# Autodesk Inventor assembly: Arm 2.0 Assembly
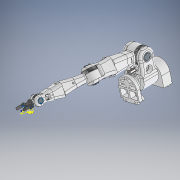
[picture p0: Inventor's stored thumbnail of the model, 180x180]
Saved by Autodesk Inventor 2017 SP1 (Build 210196100, 196)
## iProperties
Created: 2017-09-28
Part Number: Arm 2.0 Assembly
Document SubType Name: Assembly
Designer: Zach
Author: Zach
## Documents named in this file (43)
- C:\Users\Zach\Documents\GitHub\tr1\src\Body\Arm 2.0 Assembly\Arm 2.0 Assembly.iam
- C:\Users\Zach\Documents\GitHub\tr1\src\Body\Arm 2.0 Assembly\Steel Rod 8mm x 135mm.ipt
- C:\Users\Zach\Documents\GitHub\tr1\lib\22x8x8mm Bearing.ipt
- C:\Users\Zach\Documents\GitHub\tr1\src\Body\Arm 2.0 Assembly\AA004.ipt
- C:\Users\Zach\Documents\GitHub\tr1\lib\QS12MM250\QS12MM250.ipt
- C:\Users\Zach\Documents\GitHub\tr1\src\Body\Arm 2.0 Assembly\AA010.ipt
- C:\Users\Zach\Documents\GitHub\tr1\src\Body\Arm 2.0 Assembly\Steel Rod 8mm x 100mm.ipt
- C:\Users\Zach\Documents\GitHub\tr1\src\Body\Arm 2.0 Assembly\AA013.ipt
- C:\Users\Zach\Documents\GitHub\tr1\src\Body\Arm 2.0 Assembly\AA014.ipt
- C:\Users\Zach\Documents\GitHub\tr1\lib\12V DC Motor 378-1.ipt
- C:\Users\Zach\Documents\Inventor\Content Center Files\R2017\en-US\ISO 4016\ISO 4016 - M5 x 25.ipt
- C:\Users\Zach\Documents\Inventor\Content Center Files\R2017\en-US\ISO 4017(1)\ISO 4017 - M5 x 12 - ISO.ipt
- C:\Users\Zach\Documents\Inventor\Content Center Files\R2017\en-US\ISO 4017(1)\ISO 4017 - M5 x 20 - ISO.ipt
- C:\Users\Zach\Documents\GitHub\tr1\src\Body\Arm 2.0 Assembly\AA019.ipt
- C:\Users\Zach\Documents\GitHub\tr1\src\Body\Arm 2.0 Assembly\AA020.ipt
- C:\Users\Zach\Documents\GitHub\tr1\src\Body\Arm 2.0 Assembly\AA021.ipt
- C:\Users\Zach\Documents\GitHub\tr1\src\Body\Arm 2.0 Assembly\Steel Rod 8mm x 80mm.ipt
- C:\Users\Zach\Documents\GitHub\tr1\src\Body\Arm 2.0 Assembly\AA023.ipt
- C:\Users\Zach\Documents\GitHub\BCN3D-Moveo\Autodesk Inventor files\Gripper B Assembly.iam
- C:\Users\Zach\Documents\Inventor\Content Center Files\R2017\en-US\CNS 4320\CNS 4320 - M8 x 1 x 100.ipt
- C:\Users\Zach\Documents\GitHub\tr1\lib\AS 1110 - M8 x 150.ipt
- C:\Users\Zach\Documents\GitHub\tr1\lib\8mm Hub.ipt
- C:\Users\Zach\Documents\GitHub\tr1\src\Body\Arm 2.0 Assembly\Arm 2.0 Assembly\Design Accelerator\Spur Gears5.iam
- C:\Users\Zach\Documents\GitHub\tr1\lib\4mm mounting hub.ipt
- C:\Users\Zach\Documents\GitHub\tr1\lib\6201RS\6201RS.ipt
- C:\Users\Zach\Documents\GitHub\tr1\lib\U51105\U51105.ipt
- C:\Users\Zach\Documents\GitHub\tr1\src\Body\Arm 2.0 Assembly\AA033.ipt
- C:\Users\Zach\Documents\GitHub\tr1\src\Body\Arm 2.0 Assembly\AA032.ipt
- C:\Users\Zach\Documents\GitHub\tr1\src\Body\Arm 2.0 Assembly\AA031.ipt
- C:\Users\Zach\Documents\GitHub\tr1\lib\Timing Pulley - T5 4mm Bore 15mm Width.ipt
- C:\Users\Zach\Documents\GitHub\tr1\src\Body\Arm 2.0 Assembly\AA034.ipt
- C:\Users\Zach\Documents\GitHub\tr1\src\Body\Arm 2.0 Assembly\Arm 2.0 Assembly\Design Accelerator\Spur Gears6.iam
- C:\Users\Zach\Documents\GitHub\tr1\src\Body\Arm 2.0 Assembly\AA008c.ipt
- C:\Users\Zach\Documents\GitHub\tr1\src\Body\Arm 2.0 Assembly\AA008d.ipt
- C:\Users\Zach\Documents\GitHub\tr1\src\Body\Arm 2.0 Assembly\AA035.ipt
- C:\Users\Zach\Documents\GitHub\tr1\src\Body\Arm 2.0 Assembly\Arm 2.0 Assembly\Design Accelerator\Spur Gears7.iam
- C:\Users\Zach\Documents\GitHub\tr1\src\Body\Arm 2.0 Assembly\AA036.ipt
- C:\Users\Zach\Documents\GitHub\tr1\src\Body\Arm 2.0 Assembly\AA037.ipt
- C:\Users\Zach\Documents\GitHub\tr1\src\Body\Arm 2.0 Assembly\AA016b.ipt
- C:\Users\Zach\Documents\GitHub\tr1\src\Body\Arm 2.0 Assembly\AA005b.ipt
- C:\Users\Zach\Documents\GitHub\tr1\src\Body\Arm 2.0 Assembly\AA006b.ipt
- C:\Users\Zach\Documents\GitHub\tr1\src\Body\Arm 2.0 Assembly\AA001c.ipt
- C:\Users\Zach\Documents\GitHub\tr1\lib\uxcell 12V 5RPM 8mm Worm Gear Motor\uxcell 12V 5RPM 8mm Worm Gear Motor.ipt
## Components (76 placed, 40 different names)
1. AA001c:1 — Mate:554, Mate:555, Mate:556, Mate:557, Mate:558, Mate:559, Mate:560, Flush:18, Mate:561, Mate:562, Mate:563, Mate:564, Mate:565, Mate:566, Mate:567, Mate:568, Mate:569, Mate:570, Mate:571, Mate:572
2. AA004:1 — Mate:23, Mate:345, Mate:347, Mate:350, Mate:352, Mate:353, Mate:357, Mate:554, Mate:555, Mate:556
3. AA005b:1 — Mate:537, Mate:538, Mate:539, Mate:541, Mate:542, Mate:543, Mate:546
4. AA006b:1 — Mate:544, Mate:545, Mate:546
5. AA008c:1 — Mate:449, Mate:450, Mate:451, Mate:452, Mate:453, Mate:454, Mate:463, Mate:464, Mate:466, Mate:467, Mate:481, Mate:497
6. AA008d:1 — Mate:455, Mate:456, Mate:457, Mate:461, Mate:463, Mate:464, Mate:466, Mate:467, Mate:480, Mate:482
7. AA010:1 — Mate:55, Flush:6, Mate:56, Flush:7, Flush:8, Mate:64, Mate:65, Mate:66, Mate:67, Mate:68, Mate:69, Mate:486, Mate:487, Mate:488, Mate:490, Mate:492, Mate:493, Mate:494, Mate:495, Mate:496, Mate:497
8. AA013:1 — Mate:148, Mate:149, Mate:150, Mate:151, Mate:152, Mate:153, Mate:436, Mate:558, Mate:559
9. AA013:2 — Mate:142, Mate:143, Mate:144, Mate:145, Mate:146, Mate:147, Mate:563, Mate:564, Mate:565
10. AA014:1 — Mate:64, Mate:65, Mate:66, Mate:160, Mate:161, Mate:162, Mate:163, Mate:164, Mate:165
11. AA014:2 — Mate:67, Mate:68, Mate:69, Mate:154, Mate:155, Mate:156, Mate:157, Mate:158, Mate:159
12. AA016b:1 — Mate:518, Mate:519, Mate:520, Mate:521, Mate:525, Mate:526, Mate:527, Mate:529, Mate:530
13. AA019:1 — Mate:174, Mate:175, Mate:182, Mate:183, Mate:185, Flush:15, Flush:16, Flush:17, Mate:188, Mate:189, Mate:190, Mate:191, Mate:192, Mate:193, Mate:388, Mate:400, Mate:401, Mate:533, Mate:536
14. AA020:1 — Mate:171, Mate:172, Mate:173, Mate:175, Mate:194, Mate:196
15. AA021:1 — Mate:171, Mate:172, Mate:173, Mate:174, Mate:195
16. AA023:1 — Mate:188, Mate:189, Mate:193
17. AA023:2 — Mate:190, Mate:191, Mate:192
18. AA031:1 — Mate:366, Mate:367, Mate:523, Mate:524
19. AA032:2 — Mate:465
20. AA033:1 — Mate:351, Mate:352, Mate:353, Mate:355, Mate:356
21. AA034:1 — Mate:388, Mate:529, Mate:533, Mate:534, Mate:535, Mate:536
22. AA036:1 — Mate:498, Mate:500, Mate:501, Mate:502, Mate:503, Mate:511
23. AA037:1 — Mate:501, Mate:502, Mate:503, Mate:514, Mate:515, Mate:516, Mate:517, Mate:518, Mate:519, Mate:520, Mate:530
24. Gripper B Assembly:1 [sub-assembly] — Mate:194, Mate:195, Mate:196
25. 22x8x8mm Bearing:1 — Mate:433, Mate:560
26. 22x8x8mm Bearing:2 — Mate:437, Mate:562
27. 22x8x8mm Bearing:3 — Mate:55, Flush:6, Mate:57
28. 22x8x8mm Bearing:4 — Mate:56, Flush:7
29. 22x8x8mm Bearing:5 — Mate:186, Flush:16
30. 22x8x8mm Bearing:6 — Mate:187, Flush:17
31. 22x8x8mm Bearing:7 — Mate:264, Mate:526
32. 22x8x8mm Bearing:8 — Mate:527, Mate:528
33. 22x8x8mm Bearing:13 — Mate:451, Mate:452
34. 22x8x8mm Bearing:14 — Mate:449, Mate:450
35. QS12MM250:1 — Mate:23, Mate:344, Mate:346, Mate:348, Mate:351, Mate:354, Mate:484, Mate:537, Mate:544
36. Steel Rod 8mm x 135mm:1 — Mate:433, Mate:436, Mate:437, Mate:476, Mate:477, Flush:18
37. Steel Rod 8mm x 100mm:1 — Mate:57, Flush:8, Mate:491, Mate:498
38. Steel Rod 8mm x 80mm:1 — Mate:185, Flush:15, Mate:186, Mate:187
39. 12V DC Motor 378-1:2 — Mate:376, Mate:486, Mate:487, Mate:488, Mate:489
40. 12V DC Motor 378-1:3 — Mate:182, Mate:183, Mate:392, Mate:394, Mate:400
41. 12V DC Motor 378-1:4 — Mate:514, Mate:515, Mate:516, Mate:522
42. 12V DC Motor 378-1:6 — Mate:340, Mate:342, Mate:538, Mate:539, Mate:540, Mate:543
43. 12V DC Motor 378-1:7 — Mate:455, Mate:456, Mate:457, Mate:460, Mate:465
44. 6201RS:1 — Mate:346, Mate:347
45. 6201RS:2 — Mate:356, Mate:357
46. U51105:1 — Mate:348, Mate:349, Mate:542
47. U51105:2 — Mate:354, Mate:355, Mate:545
48. 8mm Hub:2 — Mate:368, Mate:531, Mate:534, Mate:535
49. 8mm Hub:3 — Mate:493, Mate:494, Mate:495
50. 4mm mounting hub:1 — Mate:340, Mate:343, Mate:540, Mate:541
51. 4mm mounting hub:3 — Mate:366, Mate:367, Mate:517, Mate:522, Mate:523, Mate:524
52. 4mm mounting hub:5 — Mate:376, Mate:513
53. 4mm mounting hub:6 — Mate:392, Mate:395, Mate:396, Mate:401
54. 4mm mounting hub:7 — Mate:460, Mate:461
55. Timing Pulley - T5 4mm Bore 15mm Width:3 — Mate:394, Mate:395, Mate:396
56. ISO 4016 M5 x 25:9
57. ISO 4016 M5 x 25:10
58. ISO 4017 M5 x 20:1 — Mate:146, Mate:147
59. ISO 4017 M5 x 20:2 — Mate:144, Mate:145
60. ISO 4017 M5 x 20:3 — Mate:142, Mate:143
61. ISO 4017 M5 x 20:4 — Mate:148, Mate:149
62. ISO 4017 M5 x 20:5 — Mate:152, Mate:153
63. ISO 4017 M5 x 20:6 — Mate:150, Mate:151
64. ISO 4017 M5 x 12:1 — Mate:154, Mate:155
65. ISO 4017 M5 x 12:2 — Mate:156, Mate:158
66. ISO 4017 M5 x 12:3 — Mate:157, Mate:159
67. ISO 4017 M5 x 12:4 — Mate:160, Mate:161
68. ISO 4017 M5 x 12:5 — Mate:162, Mate:163
69. ISO 4017 M5 x 12:6 — Mate:164, Mate:165
70. CNS 4320 M8 x 100:1 — Mate:264, Mate:368, Mate:521, Mate:525, Mate:528, Mate:531
71. AS 1110 - Metric M8 x 80:2 — Mate:453, Mate:454, Mate:496
72. Spur Gears:5 [sub-assembly] — Mate:342, Mate:343, Mate:344, Mate:345, Mate:349, Mate:350
73. Spur Gears:6 [sub-assembly] — Mate:476, Mate:478, Mate:479, Mate:566, Mate:567
74. Spur Gear2:1 — Mate:477, Mate:478, Mate:479, Mate:480, Mate:481, Mate:482, Mate:557, Mate:561
75. Spur Gears:7 [sub-assembly] — Mate:489, Mate:490, Mate:491, Mate:492, Mate:500, Mate:511, Mate:513
76. uxcell 12V 5RPM 8mm Worm Gear Motor:1 — Mate:568, Mate:569, Mate:570, Mate:571, Mate:572
## Relationships (188: Mate 181, Flush 7)
- Mate:23: AA004:1 ↔ QS12MM250:1
- Mate:55: AA010:1 ↔ 22x8x8mm Bearing:3
- Flush:6: AA010:1 ↔ 22x8x8mm Bearing:3
- Mate:56: AA010:1 ↔ 22x8x8mm Bearing:4
- Flush:7: AA010:1 ↔ 22x8x8mm Bearing:4
- Mate:57: 22x8x8mm Bearing:3 ↔ Steel Rod 8mm x 100mm:1
- Flush:8 (2.5 mm): AA010:1 ↔ Steel Rod 8mm x 100mm:1
- Mate:64: AA010:1 ↔ AA014:1
- Mate:65: AA010:1 ↔ AA014:1
- Mate:66: AA010:1 ↔ AA014:1
- Mate:67: AA010:1 ↔ AA014:2
- Mate:68: AA010:1 ↔ AA014:2
- Mate:69: AA010:1 ↔ AA014:2
- Mate:142: AA013:2 ↔ ISO 4017 M5 x 20:3
- Mate:143: AA013:2 ↔ ISO 4017 M5 x 20:3
- Mate:144: AA013:2 ↔ ISO 4017 M5 x 20:2
- Mate:145: AA013:2 ↔ ISO 4017 M5 x 20:2
- Mate:146: AA013:2 ↔ ISO 4017 M5 x 20:1
- Mate:147: AA013:2 ↔ ISO 4017 M5 x 20:1
- Mate:148: AA013:1 ↔ ISO 4017 M5 x 20:4
- Mate:149: AA013:1 ↔ ISO 4017 M5 x 20:4
- Mate:150: AA013:1 ↔ ISO 4017 M5 x 20:6
- Mate:151: AA013:1 ↔ ISO 4017 M5 x 20:6
- Mate:152: AA013:1 ↔ ISO 4017 M5 x 20:5
- Mate:153: AA013:1 ↔ ISO 4017 M5 x 20:5
- Mate:154: AA014:2 ↔ ISO 4017 M5 x 12:1
- Mate:155: AA014:2 ↔ ISO 4017 M5 x 12:1
- Mate:156: AA014:2 ↔ ISO 4017 M5 x 12:2
- Mate:157: AA014:2 ↔ ISO 4017 M5 x 12:3
- Mate:158: AA014:2 ↔ ISO 4017 M5 x 12:2
- Mate:159: AA014:2 ↔ ISO 4017 M5 x 12:3
- Mate:160: AA014:1 ↔ ISO 4017 M5 x 12:4
- Mate:161: AA014:1 ↔ ISO 4017 M5 x 12:4
- Mate:162: AA014:1 ↔ ISO 4017 M5 x 12:5
- Mate:163: AA014:1 ↔ ISO 4017 M5 x 12:5
- Mate:164: AA014:1 ↔ ISO 4017 M5 x 12:6
- Mate:165: AA014:1 ↔ ISO 4017 M5 x 12:6
- Mate:171: AA020:1 ↔ AA021:1
- Mate:172: AA020:1 ↔ AA021:1
- Mate:173: AA020:1 ↔ AA021:1
- Mate:174 (1 mm): AA019:1 ↔ AA021:1
- Mate:175: AA019:1 ↔ AA020:1
- Mate:182: AA019:1 ↔ 12V DC Motor 378-1:3
- Mate:183: AA019:1 ↔ 12V DC Motor 378-1:3
- Mate:185: AA019:1 ↔ Steel Rod 8mm x 80mm:1
- Flush:15: AA019:1 ↔ Steel Rod 8mm x 80mm:1
- Mate:186: 22x8x8mm Bearing:5 ↔ Steel Rod 8mm x 80mm:1
- Flush:16: AA019:1 ↔ 22x8x8mm Bearing:5
- Mate:187: 22x8x8mm Bearing:6 ↔ Steel Rod 8mm x 80mm:1
- Flush:17: AA019:1 ↔ 22x8x8mm Bearing:6
- Mate:188: AA019:1 ↔ AA023:1
- Mate:189: AA019:1 ↔ AA023:1
- Mate:190: AA019:1 ↔ AA023:2
- Mate:191: AA019:1 ↔ AA023:2
- Mate:192: AA019:1 ↔ AA023:2
- Mate:193: AA019:1 ↔ AA023:1
- Mate:194: AA020:1 ↔ Gripper B Assembly:1
- Mate:195: AA021:1 ↔ Gripper B Assembly:1
- Mate:196: AA020:1 ↔ Gripper B Assembly:1
- Mate:264: 22x8x8mm Bearing:7 ↔ CNS 4320 M8 x 100:1
- Mate:340: 12V DC Motor 378-1:6 ↔ 4mm mounting hub:1
- Mate:342: 12V DC Motor 378-1:6 ↔ Spur Gears:5
- Mate:343: 4mm mounting hub:1 ↔ Spur Gears:5
- Mate:344: QS12MM250:1 ↔ Spur Gears:5
- Mate:345: AA004:1 ↔ Spur Gears:5
- Mate:346: QS12MM250:1 ↔ 6201RS:1
- Mate:347: AA004:1 ↔ 6201RS:1
- Mate:348: QS12MM250:1 ↔ U51105:1
- Mate:349: U51105:1 ↔ Spur Gears:5
- Mate:350: AA004:1 ↔ Spur Gears:5
- Mate:351: AA033:1 ↔ QS12MM250:1
- Mate:352: AA004:1 ↔ AA033:1
- Mate:353: AA004:1 ↔ AA033:1
- Mate:354: QS12MM250:1 ↔ U51105:2
- Mate:355: AA033:1 ↔ U51105:2
- Mate:356: AA033:1 ↔ 6201RS:2
- Mate:357: AA004:1 ↔ 6201RS:2
- Mate:366: AA031:1 ↔ 4mm mounting hub:3
- Mate:367: AA031:1 ↔ 4mm mounting hub:3
- Mate:368: 8mm Hub:2 ↔ CNS 4320 M8 x 100:1
- Mate:376: 12V DC Motor 378-1:2 ↔ 4mm mounting hub:5
- Mate:388: AA019:1 ↔ AA034:1
- Mate:392: 12V DC Motor 378-1:3 ↔ 4mm mounting hub:6
- Mate:394: 12V DC Motor 378-1:3 ↔ Timing Pulley - T5 4mm Bore 15mm Width:3
- Mate:395: 4mm mounting hub:6 ↔ Timing Pulley - T5 4mm Bore 15mm Width:3
- Mate:396: 4mm mounting hub:6 ↔ Timing Pulley - T5 4mm Bore 15mm Width:3
- Mate:400: AA019:1 ↔ 12V DC Motor 378-1:3
- Mate:401: AA019:1 ↔ 4mm mounting hub:6
- Mate:433: 22x8x8mm Bearing:1 ↔ Steel Rod 8mm x 135mm:1
- Mate:436: AA013:1 ↔ Steel Rod 8mm x 135mm:1
- Mate:437: 22x8x8mm Bearing:2 ↔ Steel Rod 8mm x 135mm:1
- Mate:449: AA008c:1 ↔ 22x8x8mm Bearing:14
- Mate:450: AA008c:1 ↔ 22x8x8mm Bearing:14
- Mate:451: AA008c:1 ↔ 22x8x8mm Bearing:13
- Mate:452: AA008c:1 ↔ 22x8x8mm Bearing:13
- Mate:453: AA008c:1 ↔ AS 1110 - Metric M8 x 80:2
- Mate:454: AA008c:1 ↔ AS 1110 - Metric M8 x 80:2
- Mate:455: AA008d:1 ↔ 12V DC Motor 378-1:7
- Mate:456: AA008d:1 ↔ 12V DC Motor 378-1:7
- Mate:457: AA008d:1 ↔ 12V DC Motor 378-1:7
- [Mate]: AA032:2 ↔ 4mm mounting hub:7
- [Mate]: AA032:2 ↔ 4mm mounting hub:7
- Mate:460: 12V DC Motor 378-1:7 ↔ 4mm mounting hub:7
- Mate:461: AA008d:1 ↔ 4mm mounting hub:7
- Mate:463: AA008c:1 ↔ AA008d:1
- Mate:464: AA008c:1 ↔ AA008d:1
- Mate:465: AA032:2 ↔ 12V DC Motor 378-1:7
- Mate:466: AA008c:1 ↔ AA008d:1
- Mate:467: AA008c:1 ↔ AA008d:1
- Mate:476: Steel Rod 8mm x 135mm:1 ↔ Spur Gears:6
- Mate:477: Steel Rod 8mm x 135mm:1 ↔ Spur Gear2:1
- Mate:478: Spur Gears:6 ↔ Spur Gear2:1
- Mate:479: Spur Gears:6 ↔ Spur Gear2:1
- Mate:480: AA008d:1 ↔ Spur Gear2:1
- Mate:481: AA008c:1 ↔ Spur Gear2:1
- Mate:482: AA008d:1 ↔ Spur Gear2:1
- Mate:484: QS12MM250:1
- Mate:486: AA010:1 ↔ 12V DC Motor 378-1:2
- Mate:487: AA010:1 ↔ 12V DC Motor 378-1:2
- Mate:488: AA010:1 ↔ 12V DC Motor 378-1:2
- Mate:489: 12V DC Motor 378-1:2 ↔ Spur Gears:7
- Mate:490: AA010:1 ↔ Spur Gears:7
- Mate:491: Steel Rod 8mm x 100mm:1 ↔ Spur Gears:7
- Mate:492: AA010:1 ↔ Spur Gears:7
- Mate:493: AA010:1 ↔ 8mm Hub:3
- Mate:494: AA010:1 ↔ 8mm Hub:3
- Mate:495: AA010:1 ↔ 8mm Hub:3
- Mate:496: AA010:1 ↔ AS 1110 - Metric M8 x 80:2
- Mate:497: AA008c:1 ↔ AA010:1
- Mate:498: AA036:1 ↔ Steel Rod 8mm x 100mm:1
- Mate:500: AA036:1 ↔ Spur Gears:7
- Mate:501: AA036:1 ↔ AA037:1
- Mate:502: AA036:1 ↔ AA037:1
- Mate:503: AA036:1 ↔ AA037:1
- Mate:511: AA036:1 ↔ Spur Gears:7
- Mate:513: 4mm mounting hub:5 ↔ Spur Gears:7
- Mate:514: AA037:1 ↔ 12V DC Motor 378-1:4
- Mate:515: AA037:1 ↔ 12V DC Motor 378-1:4
- Mate:516: AA037:1 ↔ 12V DC Motor 378-1:4
- Mate:517: AA037:1 ↔ 4mm mounting hub:3
- Mate:518: AA016b:1 ↔ AA037:1
- Mate:519: AA016b:1 ↔ AA037:1
- Mate:520: AA016b:1 ↔ AA037:1
- Mate:521: AA016b:1 ↔ CNS 4320 M8 x 100:1
- Mate:522: 12V DC Motor 378-1:4 ↔ 4mm mounting hub:3
- Mate:523: AA031:1 ↔ 4mm mounting hub:3
- Mate:524: AA031:1 ↔ 4mm mounting hub:3
- Mate:525: AA016b:1 ↔ CNS 4320 M8 x 100:1
- Mate:526 (0.5 mm): AA016b:1 ↔ 22x8x8mm Bearing:7
- Mate:527 (0.5 mm): AA016b:1 ↔ 22x8x8mm Bearing:8
- Mate:528: 22x8x8mm Bearing:8 ↔ CNS 4320 M8 x 100:1
- Mate:529: AA016b:1 ↔ AA034:1
- Mate:530: AA016b:1 ↔ AA037:1
- Mate:531: 8mm Hub:2 ↔ CNS 4320 M8 x 100:1
- Mate:533: AA019:1 ↔ AA034:1
- Mate:534: AA034:1 ↔ 8mm Hub:2
- Mate:535: AA034:1 ↔ 8mm Hub:2
- Mate:536: AA019:1 ↔ AA034:1
- Mate:537: AA005b:1 ↔ QS12MM250:1
- Mate:538: AA005b:1 ↔ 12V DC Motor 378-1:6
- Mate:539: AA005b:1 ↔ 12V DC Motor 378-1:6
- Mate:540: 12V DC Motor 378-1:6 ↔ 4mm mounting hub:1
- Mate:541: AA005b:1 ↔ 4mm mounting hub:1
- Mate:542: AA005b:1 ↔ U51105:1
- Mate:543: AA005b:1 ↔ 12V DC Motor 378-1:6
- Mate:544: AA006b:1 ↔ QS12MM250:1
- Mate:545: AA006b:1 ↔ U51105:2
- Mate:546: AA005b:1 ↔ AA006b:1
- Mate:554: AA001c:1 ↔ AA004:1
- Mate:555: AA001c:1 ↔ AA004:1
- Mate:556: AA001c:1 ↔ AA004:1
- Mate:557: AA001c:1 ↔ Spur Gear2:1
- Mate:558: AA001c:1 ↔ AA013:1
- Mate:559: AA001c:1 ↔ AA013:1
- Mate:560: AA001c:1 ↔ 22x8x8mm Bearing:1
- Flush:18: AA001c:1 ↔ Steel Rod 8mm x 135mm:1
- Mate:561 (2.25 mm): AA001c:1 ↔ Spur Gear2:1
- Mate:562: AA001c:1 ↔ 22x8x8mm Bearing:2
- Mate:563: AA001c:1 ↔ AA013:2
- Mate:564: AA001c:1 ↔ AA013:2
- Mate:565: AA001c:1 ↔ AA013:2
- Mate:566: AA001c:1 ↔ Spur Gears:6
- Mate:567 (1 mm): AA001c:1 ↔ Spur Gears:6
- Mate:568: AA001c:1 ↔ uxcell 12V 5RPM 8mm Worm Gear Motor:1
- Mate:569: AA001c:1 ↔ uxcell 12V 5RPM 8mm Worm Gear Motor:1
- Mate:570: AA001c:1 ↔ uxcell 12V 5RPM 8mm Worm Gear Motor:1
- Mate:571: AA001c:1 ↔ uxcell 12V 5RPM 8mm Worm Gear Motor:1
- Mate:572: AA001c:1 ↔ uxcell 12V 5RPM 8mm Worm Gear Motor:1
## Named parameters: d576_d462 = 0 mm, d577_d463 = 0 mm
